# Autodesk Inventor assembly: 000 ASY GBK Gubkinskiy
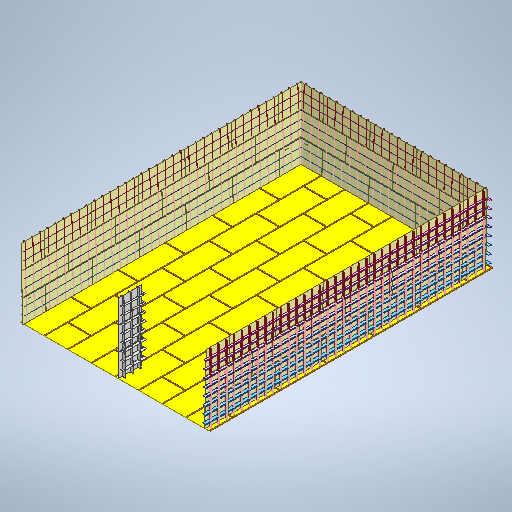
[picture p0: Inventor's stored thumbnail of the model, 512x512]
Saved by Autodesk Inventor 2026 (Build 300175000, 175)
## iProperties
Created: 2026-04-17
Part Number: 000 ASY GBK Gubkinskiy
Document SubType Name: Assembly
Designer: admin
Mass: 2.02017e+07 g
Surface Area: 1.30705e+07 cm^2
Volume: 2.57346e+06 cm^3
Density: 7.85 g/cm^3
Author: admin
## Documents named in this file (11)
- C:\Users\pokla\Documents\Inventor\GBK-Gubkinskiy\000 ASY GBK Gubkinskiy.iam
- C:\Users\pokla\Documents\Inventor\GBK-Gubkinskiy\GBK bottom.ipt
- C:\Users\pokla\Documents\Inventor\GBK-Gubkinskiy\GBK dummy wall 1.ipt
- C:\Users\pokla\Documents\Inventor\GBK-Gubkinskiy\GBK dummy wall 4.ipt
- C:\Users\pokla\Documents\Inventor\GBK-Gubkinskiy\GBK overall model.ipt
- C:\Users\pokla\Documents\Inventor\GBK-Gubkinskiy\ASY GBK 3110 wall shield Center 1.iam
- C:\Users\pokla\Documents\Inventor\GBK-Gubkinskiy\ASY GBK 3210 wall shield Center 3.iam
- C:\Users\pokla\Documents\Inventor\GBK-Gubkinskiy\ASY GBK 3310 wall shield Center 4.iam
- C:\Users\pokla\Documents\Inventor\GBK-Gubkinskiy\ASY GBK правая стенка.iam
- C:\Users\pokla\Documents\Inventor\GBK-Gubkinskiy\ASY GBK предварительная торцевая.iam
- C:\Users\pokla\Documents\Inventor\GBK-Gubkinskiy\090 ASY bottom.iam
## Components (13 placed, 10 different names)
1. GBK bottom.ipt:1 — Совмещение:10, Совмещение:11, Совмещение:12, Совмещение:13, Совмещение:14, Жесткий:1, Заподлицо:4, Заподлицо:6, Заподлицо:7, Заподлицо:8
2. GBK dummy wall 1.ipt:1 — Совмещение:10
3. GBK dummy wall 1.ipt:2 — Совмещение:11, Совмещение:12
4. GBK dummy wall 4.ipt:1 — Совмещение:13, Совмещение:14
5. GBK overall model.ipt:1 — Жесткий:1
6. ASY GBK правая стенка.iam:1 [sub-assembly]
7. ASY GBK предварительная торцевая.iam:1 [sub-assembly]
8. ASY GBK предварительная торцевая.iam:2 [sub-assembly] — Совмещение:17, Заподлицо:4
9. ASY GBK правая стенка.iam:2 [sub-assembly] — Заподлицо:5, Заподлицо:6
10. 0701 ASY GBK wall shield Center 4.iam:1 [sub-assembly] — Жесткий:2, Жесткий:3
11. 01001 ASY GBK wall shield Center 10.iam:1 [sub-assembly] — Жесткий:3
12. 0401 ASY GBK wall shield Center 1.iam:1 [sub-assembly] — Жесткий:2, Совмещение:18, Заподлицо:7
13. 090 ASY bottom.iam:1 [sub-assembly] — Совмещение:19, Заподлицо:8
## Relationships (20: Mate 10, Flush 7, WeldJoint 3)
- [Flush]: GBK bottom.ipt:1 ↔ ASY GBK правая стенка.iam:1
- [Mate]: GBK bottom.ipt:1 ↔ ASY GBK правая стенка.iam:1
- Совмещение:10 [Mate]: GBK bottom.ipt:1 ↔ GBK dummy wall 1.ipt:1
- Совмещение:11 [Mate]: GBK bottom.ipt:1 ↔ GBK dummy wall 1.ipt:2
- Совмещение:12 [Mate]: GBK bottom.ipt:1 ↔ GBK dummy wall 1.ipt:2
- Совмещение:13 [Mate]: GBK bottom.ipt:1 ↔ GBK dummy wall 4.ipt:1
- Совмещение:14 [Mate]: GBK bottom.ipt:1 ↔ GBK dummy wall 4.ipt:1
- Жесткий:1 [WeldJoint]: GBK bottom.ipt:1 ↔ GBK overall model.ipt:1
- [Mate]: ASY GBK предварительная торцевая.iam:1
- [Flush]: GBK bottom.ipt:1 ↔ ASY GBK предварительная торцевая.iam:1
- Совмещение:17 [Mate]: ASY GBK предварительная торцевая.iam:2
- Заподлицо:4 [Flush]: GBK bottom.ipt:1 ↔ ASY GBK предварительная торцевая.iam:2
- Заподлицо:5 [Flush]: ASY GBK правая стенка.iam:2
- Заподлицо:6 [Flush]: GBK bottom.ipt:1 ↔ ASY GBK правая стенка.iam:2
- Жесткий:2 [WeldJoint]: 0701 ASY GBK wall shield Center 4.iam:1 ↔ 0401 ASY GBK wall shield Center 1.iam:1
- Жесткий:3 [WeldJoint]: 0701 ASY GBK wall shield Center 4.iam:1 ↔ 01001 ASY GBK wall shield Center 10.iam:1
- Совмещение:18 [Mate]: 0401 ASY GBK wall shield Center 1.iam:1
- Заподлицо:7 [Flush]: GBK bottom.ipt:1 ↔ 0401 ASY GBK wall shield Center 1.iam:1
- Совмещение:19 [Mate]: 090 ASY bottom.iam:1
- Заподлицо:8 [Flush]: GBK bottom.ipt:1 ↔ 090 ASY bottom.iam:1
## Named parameters: Зазор_по_горизонту = 1 mm, d120_Зазор_по_горизонту = 1 mm, d141_Зазор_по_горизонту = 1 mm, d159_d141_Зазор_по_горизонту = 1 mm, d175_d141_Зазор_по_горизонту = 1 mm
